# Autodesk Inventor assembly: 車体
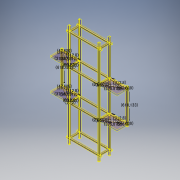
[picture p0: Inventor's stored thumbnail of the model, 180x180]
Saved by Autodesk Inventor 2018 (Build 220112000, 112)
## iProperties
Created: 2017-09-13
Part Number: 車体
Material: 一般
Document SubType Name: Assembly
Designer: mura5
Author: mura5
## Documents named in this file (8)
- C:\Users\Katsunari Murase\Documents\rbbr\cart\シャーシ改\車体.iam
- C:\Users\Katsunari Murase\Documents\rbbr\cart\シャーシ改\Pipe1.ipt
- C:\Users\Katsunari Murase\Documents\rbbr\cart\シャーシ改\Pipe2.ipt
- C:\Users\Katsunari Murase\Documents\rbbr\cart\シャーシ改\Pipe3.ipt
- C:\Users\Katsunari Murase\Documents\rbbr\cart\シャーシ改\Pipe4.ipt
- C:\Users\Katsunari Murase\Documents\rbbr\cart\シャーシ改\Pipe5.ipt
- C:\Users\Katsunari Murase\Documents\rbbr\cart\シャーシ改\Pipe6.ipt
- C:\Users\Katsunari Murase\Documents\rbbr\cart\シャーシ改\Pipe7.ipt
## Components (30 placed, 7 different names)
1. Pipe1:1 — フラッシュ:1, 回転:1, メイト:1, フラッシュ:4, メイト:2, フラッシュ:5, メイト:9, フラッシュ:15, メイト:10, フラッシュ:16, メイト:11, フラッシュ:18, メイト:12, フラッシュ:21, メイト:18, フラッシュ:35, フラッシュ:38, メイト:19
2. Pipe1:2 — フラッシュ:2, 回転:2, フラッシュ:3, 回転:3, メイト:5, フラッシュ:6, メイト:6, フラッシュ:8, メイト:7, フラッシュ:11, メイト:8, フラッシュ:12, メイト:16, メイト:17, フラッシュ:32, フラッシュ:34
3. Pipe2:1 — フラッシュ:1, 回転:1, フラッシュ:2, 回転:2, メイト:4, フラッシュ:7, フラッシュ:14
4. Pipe2:2 — フラッシュ:3, 回転:3, フラッシュ:13, フラッシュ:20, メイト:30
5. Pipe3:1 — メイト:1, フラッシュ:4, メイト:4, フラッシュ:9, フラッシュ:17, フラッシュ:31, フラッシュ:36
6. Pipe3:2 — メイト:2, フラッシュ:5, フラッシュ:10, フラッシュ:19, フラッシュ:33, フラッシュ:37, メイト:30
7. Pipe4:1 — メイト:5, フラッシュ:6, フラッシュ:7, メイト:13, フラッシュ:23, フラッシュ:24
8. Pipe4:2 — メイト:6, フラッシュ:8, フラッシュ:9
9. Pipe4:3 — メイト:7, フラッシュ:10, フラッシュ:11
10. Pipe4:4 — メイト:8, フラッシュ:12, フラッシュ:13
11. Pipe4:5 — メイト:9, フラッシュ:14, フラッシュ:15
12. Pipe4:6 — メイト:10, フラッシュ:16, フラッシュ:17, フラッシュ:30
13. Pipe4:7 — メイト:11, フラッシュ:18, フラッシュ:19, フラッシュ:28
14. Pipe4:8 — メイト:12, フラッシュ:20, フラッシュ:21
15. Pipe1:3 — フラッシュ:26, 回転:6, メイト:14, フラッシュ:27, メイト:15, フラッシュ:29, メイト:27, メイト:29
16. Pipe1:4 — メイト:13, フラッシュ:22, 回転:4, フラッシュ:23, フラッシュ:25, 回転:5, メイト:23, メイト:25
17. Pipe2:3 — フラッシュ:22, 回転:4, フラッシュ:24
18. Pipe2:4 — フラッシュ:25, 回転:5, フラッシュ:26, 回転:6
19. Pipe3:3 — メイト:14, フラッシュ:27, フラッシュ:28
20. Pipe3:4 — メイト:15, フラッシュ:29, フラッシュ:30
21. Pipe5:1 — メイト:16, フラッシュ:31, フラッシュ:32, メイト:20, フラッシュ:39, フラッシュ:40, メイト:22, フラッシュ:43
22. Pipe5:2 — メイト:17, フラッシュ:33, フラッシュ:34, メイト:24, フラッシュ:44
23. Pipe5:3 — フラッシュ:37, フラッシュ:38, メイト:19, フラッシュ:46
24. Pipe5:4 — メイト:18, フラッシュ:35, フラッシュ:36, メイト:21, フラッシュ:41, フラッシュ:42, メイト:26, フラッシュ:45
25. Pipe6:1 — メイト:20, フラッシュ:39, フラッシュ:40
26. Pipe6:2 — メイト:21, フラッシュ:41, フラッシュ:42, メイト:28
27. Pipe7:1 — メイト:22, メイト:23, フラッシュ:43
28. Pipe7:2 — メイト:24, メイト:25, フラッシュ:44
29. Pipe7:3 — メイト:26, メイト:27, フラッシュ:45
30. Pipe7:4 — メイト:28, メイト:29, フラッシュ:46
## Relationships (81: Flush 46, Mate 29, RevoluteJoint 6)
- フラッシュ:1 [Flush]: Pipe1:1 ↔ Pipe2:1
- 回転:1 [RevoluteJoint]: Pipe1:1 ↔ Pipe2:1
- フラッシュ:2 [Flush]: Pipe1:2 ↔ Pipe2:1
- 回転:2 [RevoluteJoint]: Pipe1:2 ↔ Pipe2:1
- フラッシュ:3 [Flush]: Pipe1:2 ↔ Pipe2:2
- 回転:3 [RevoluteJoint]: Pipe1:2 ↔ Pipe2:2
- メイト:1 [Mate]: Pipe1:1 ↔ Pipe3:1
- フラッシュ:4 [Flush]: Pipe1:1 ↔ Pipe3:1
- メイト:2 [Mate]: Pipe1:1 ↔ Pipe3:2
- フラッシュ:5 [Flush]: Pipe1:1 ↔ Pipe3:2
- メイト:4 [Mate] (590.9333 mm): Pipe2:1 ↔ Pipe3:1
- メイト:5 [Mate]: Pipe1:2 ↔ Pipe4:1
- フラッシュ:6 [Flush]: Pipe1:2 ↔ Pipe4:1
- フラッシュ:7 [Flush]: Pipe2:1 ↔ Pipe4:1
- メイト:6 [Mate]: Pipe1:2 ↔ Pipe4:2
- フラッシュ:8 [Flush]: Pipe1:2 ↔ Pipe4:2
- フラッシュ:9 [Flush]: Pipe3:1 ↔ Pipe4:2
- メイト:7 [Mate]: Pipe1:2 ↔ Pipe4:3
- フラッシュ:10 [Flush]: Pipe3:2 ↔ Pipe4:3
- フラッシュ:11 [Flush]: Pipe1:2 ↔ Pipe4:3
- メイト:8 [Mate]: Pipe1:2 ↔ Pipe4:4
- フラッシュ:12 [Flush]: Pipe1:2 ↔ Pipe4:4
- フラッシュ:13 [Flush]: Pipe2:2 ↔ Pipe4:4
- メイト:9 [Mate]: Pipe1:1 ↔ Pipe4:5
- フラッシュ:14 [Flush]: Pipe2:1 ↔ Pipe4:5
- フラッシュ:15 [Flush]: Pipe1:1 ↔ Pipe4:5
- メイト:10 [Mate]: Pipe1:1 ↔ Pipe4:6
- フラッシュ:16 [Flush]: Pipe1:1 ↔ Pipe4:6
- フラッシュ:17 [Flush]: Pipe3:1 ↔ Pipe4:6
- メイト:11 [Mate]: Pipe1:1 ↔ Pipe4:7
- フラッシュ:18 [Flush]: Pipe1:1 ↔ Pipe4:7
- フラッシュ:19 [Flush]: Pipe3:2 ↔ Pipe4:7
- メイト:12 [Mate]: Pipe1:1 ↔ Pipe4:8
- フラッシュ:20 [Flush]: Pipe2:2 ↔ Pipe4:8
- フラッシュ:21 [Flush]: Pipe1:1 ↔ Pipe4:8
- メイト:13 [Mate]: Pipe4:1 ↔ Pipe1:4
- フラッシュ:22 [Flush]: Pipe1:4 ↔ Pipe2:3
- 回転:4 [RevoluteJoint]: Pipe1:4 ↔ Pipe2:3
- フラッシュ:23 [Flush]: Pipe4:1 ↔ Pipe1:4
- フラッシュ:24 [Flush]: Pipe4:1 ↔ Pipe2:3
- フラッシュ:25 [Flush]: Pipe1:4 ↔ Pipe2:4
- 回転:5 [RevoluteJoint]: Pipe1:4 ↔ Pipe2:4
- フラッシュ:26 [Flush]: Pipe1:3 ↔ Pipe2:4
- 回転:6 [RevoluteJoint]: Pipe1:3 ↔ Pipe2:4
- メイト:14 [Mate]: Pipe1:3 ↔ Pipe3:3
- フラッシュ:27 [Flush]: Pipe1:3 ↔ Pipe3:3
- フラッシュ:28 [Flush]: Pipe4:7 ↔ Pipe3:3
- メイト:15 [Mate]: Pipe1:3 ↔ Pipe3:4
- フラッシュ:29 [Flush]: Pipe1:3 ↔ Pipe3:4
- フラッシュ:30 [Flush]: Pipe4:6 ↔ Pipe3:4
- メイト:16 [Mate]: Pipe1:2 ↔ Pipe5:1
- メイト:17 [Mate]: Pipe1:2 ↔ Pipe5:2
- フラッシュ:31 [Flush]: Pipe3:1 ↔ Pipe5:1
- フラッシュ:32 [Flush]: Pipe1:2 ↔ Pipe5:1
- フラッシュ:33 [Flush]: Pipe3:2 ↔ Pipe5:2
- フラッシュ:34 [Flush]: Pipe1:2 ↔ Pipe5:2
- メイト:18 [Mate]: Pipe1:1 ↔ Pipe5:4
- フラッシュ:35 [Flush]: Pipe1:1 ↔ Pipe5:4
- フラッシュ:36 [Flush]: Pipe3:1 ↔ Pipe5:4
- フラッシュ:37 [Flush]: Pipe3:2 ↔ Pipe5:3
- フラッシュ:38 [Flush]: Pipe1:1 ↔ Pipe5:3
- メイト:19 [Mate]: Pipe1:1 ↔ Pipe5:3
- メイト:20 [Mate]: Pipe5:1 ↔ Pipe6:1
- フラッシュ:39 [Flush]: Pipe5:1 ↔ Pipe6:1
- フラッシュ:40 [Flush]: Pipe5:1 ↔ Pipe6:1
- メイト:21 [Mate]: Pipe5:4 ↔ Pipe6:2
- フラッシュ:41 [Flush]: Pipe5:4 ↔ Pipe6:2
- フラッシュ:42 [Flush]: Pipe5:4 ↔ Pipe6:2
- メイト:22 [Mate]: Pipe5:1 ↔ Pipe7:1
- メイト:23 [Mate]: Pipe1:4 ↔ Pipe7:1
- フラッシュ:43 [Flush]: Pipe5:1 ↔ Pipe7:1
- メイト:24 [Mate]: Pipe5:2 ↔ Pipe7:2
- メイト:25 [Mate]: Pipe1:4 ↔ Pipe7:2
- フラッシュ:44 [Flush]: Pipe5:2 ↔ Pipe7:2
- メイト:26 [Mate]: Pipe5:4 ↔ Pipe7:3
- メイト:27 [Mate]: Pipe1:3 ↔ Pipe7:3
- フラッシュ:45 [Flush]: Pipe5:4 ↔ Pipe7:3
- メイト:28 [Mate]: Pipe6:2 ↔ Pipe7:4
- メイト:29 [Mate]: Pipe1:3 ↔ Pipe7:4
- フラッシュ:46 [Flush]: Pipe5:3 ↔ Pipe7:4
- メイト:30 [Mate] (590.9333 mm): Pipe2:2 ↔ Pipe3:2
